# Autodesk Inventor assembly: PulleySystem 1
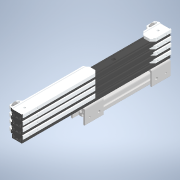
[picture p0: Inventor's stored thumbnail of the model, 180x180]
Saved by Autodesk Inventor 2020.2 (Build 242310000, 310)
## iProperties
Created: 2020-02-03
Part Number: PulleySystem 1
Document SubType Name: Assembly
Designer: maple
Author: maple
## Documents named in this file (4)
- C:\Users\AOFUser\Documents\GitHub\CAD\Robotics 2019-2020\PulleySystem\PulleySystem Final.iam
- C:\Users\AOFUser\Documents\GitHub\CAD\Robotics 2019-2020\PulleySystem\PulleySystem Part 1.ipt
- C:\Users\AOFUser\Documents\GitHub\CAD\Robotics 2019-2020\PulleySystem\1inchExtrusion.ipt
- C:\Users\AOFUser\Documents\GitHub\CAD\Robotics 2019-2020\PulleySystem\Long Robotics Mount V2.ipt
## Components (7 placed, 3 different names)
1. PulleySystem Part 1:1 — Rotational:3
2. PulleySystem Part 1:2 — Rotational:2, Rotational:3
3. PulleySystem Part 1:3 — Rotational:1, Rotational:2
4. PulleySystem Part 1:4 — Rotational:1, Rotational:4, Rotational:5
5. 1inchExtrusion:1 — Mate:1
6. Long Robotics Mount V2:1 — Rotational:5
7. Long Robotics Mount V2:2 — Rotational:4, Mate:1
## Relationships (6: RevoluteJoint 5, Mate 1)
- Rotational:1 [RevoluteJoint]: PulleySystem Part 1:3 ↔ PulleySystem Part 1:4
- Rotational:2 [RevoluteJoint]: PulleySystem Part 1:2 ↔ PulleySystem Part 1:3
- Rotational:3 [RevoluteJoint]: PulleySystem Part 1:1 ↔ PulleySystem Part 1:2
- Rotational:4 [RevoluteJoint]: PulleySystem Part 1:4 ↔ Long Robotics Mount V2:2
- Rotational:5 [RevoluteJoint]: PulleySystem Part 1:4 ↔ Long Robotics Mount V2:1
- Mate:1: 1inchExtrusion:1 ↔ Long Robotics Mount V2:2
